# Autodesk Inventor assembly: ASY DMF 01 20 snout
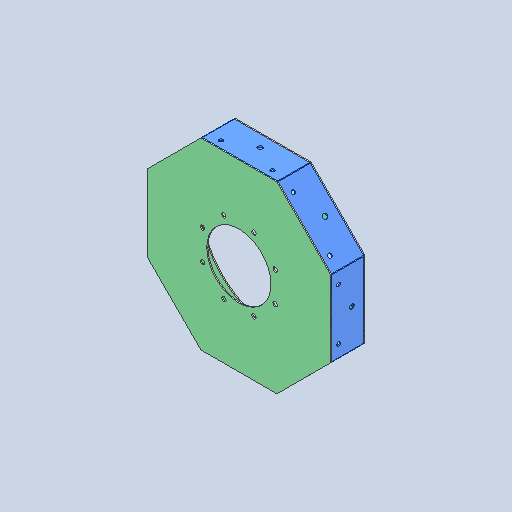
[picture p0: Inventor's stored thumbnail of the model, 512x512]
Saved by Autodesk Inventor 2026.2 (Build 302298000, 298)
## iProperties
Created: 2026-05-29
Part Number: ASY DMF 01 20 snout
Document SubType Name: Assembly
Designer: admin
Author: admin
## Documents named in this file (4)
- C:\Users\admin\Documents\Inventor\DMF-Disk-Micro-Filter\Барабан v2.1\ASY DMF 01 20 snout.iam
- C:\Users\admin\Documents\Inventor\DMF-Disk-Micro-Filter\Барабан v2.1\DMF 01 15 drum sheet 1.ipt
- C:\Users\admin\Documents\Inventor\DMF-Disk-Micro-Filter\Барабан v2.1\DMF 01 21 Барабан торец НОС v2.1.ipt
- C:\Users\admin\Documents\Inventor\DMF-Disk-Micro-Filter\Барабан v2.1\DMF 01 21 Барабан торец НОС v2.1_наруж.ipt
## Components (10 placed, 4 different names)
1. DMF 01 15 drum sheet 1.ipt:1
2. DMF 01 21 Барабан торец НОС v2.1:1
3. DMF 01 15 drum sheet 1:2
4. DMF 01 21 Барабан торец НОС v2.1_наруж:1
5. DMF 01 15 drum sheet 1:3
6. DMF 01 15 drum sheet 1:4
7. DMF 01 15 drum sheet 1:5
8. DMF 01 15 drum sheet 1:6
9. DMF 01 15 drum sheet 1:7
10. DMF 01 15 drum sheet 1:8
## Relationships (9: WeldJoint 9)
- [WeldJoint]: DMF 01 15 drum sheet 1.ipt:1 ↔ DMF 01 21 Барабан торец НОС v2.1:1
- [WeldJoint]: DMF 01 21 Барабан торец НОС v2.1:1 ↔ DMF 01 15 drum sheet 1:2
- [WeldJoint]: DMF 01 15 drum sheet 1.ipt:1 ↔ DMF 01 21 Барабан торец НОС v2.1_наруж:1
- [WeldJoint]: DMF 01 21 Барабан торец НОС v2.1:1 ↔ DMF 01 15 drum sheet 1:3
- [WeldJoint]: DMF 01 21 Барабан торец НОС v2.1:1 ↔ DMF 01 15 drum sheet 1:4
- [WeldJoint]: DMF 01 21 Барабан торец НОС v2.1:1 ↔ DMF 01 15 drum sheet 1:5
- [WeldJoint]: DMF 01 21 Барабан торец НОС v2.1:1 ↔ DMF 01 15 drum sheet 1:8
- [WeldJoint]: DMF 01 21 Барабан торец НОС v2.1:1 ↔ DMF 01 15 drum sheet 1:6
- [WeldJoint]: DMF 01 21 Барабан торец НОС v2.1:1 ↔ DMF 01 15 drum sheet 1:7
